# Autodesk Inventor assembly: Assembly1.ipt
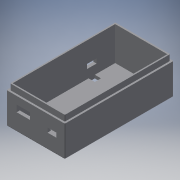
[picture p0: Inventor's stored thumbnail of the model, 180x180]
Saved by Autodesk Inventor 2019.3 (Build 233278000, 278)
## iProperties
Created: 2019-04-11
Part Number: Assembly1.ipt
Document SubType Name: Assembly
Designer: grego
Author: grego
## Documents named in this file (3)
- D:\OneDrive - njit.edu\ECE 414-001\CAD model\Half Box Correct.iam
- D:\OneDrive - njit.edu\ECE 414-001\CAD model\Smart Lock Box Middle Correct.ipt
- D:\OneDrive - njit.edu\ECE 414-001\CAD model\Smart Lock Box Bottom Correct.ipt
## Components (2 placed, 2 different names)
1. Smart Lock Box Middle Correct:1 — Flush:1, Flush:2, Mate:1
2. Smart Lock Box Bottom Correct:1 — Flush:1, Flush:2, Mate:1
## Relationships (3: Flush 2, Mate 1)
- Flush:1: Smart Lock Box Middle Correct:1 ↔ Smart Lock Box Bottom Correct:1
- Flush:2: Smart Lock Box Middle Correct:1 ↔ Smart Lock Box Bottom Correct:1
- Mate:1: Smart Lock Box Middle Correct:1 ↔ Smart Lock Box Bottom Correct:1
